# Autodesk Inventor assembly: ASY Disk Micro filter v2.0
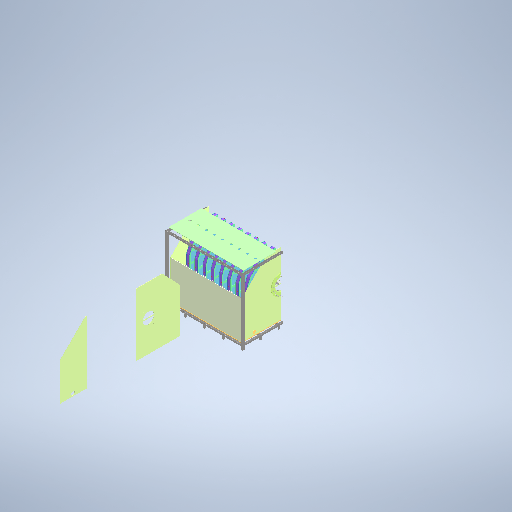
[picture p0: Inventor's stored thumbnail of the model, 512x512]
Saved by Autodesk Inventor 2025 (Build 290162010, 162A)
## iProperties
Created: 2023-08-31
Part Number: ASY Disk Micro filter v2.0
Document SubType Name: Assembly
Designer: admin
Stock Number: Дисковый_Фильтр
Author: admin
## Documents named in this file (29)
- C:\Users\pokla\Documents\Inventor\ДФО\ДМФ\DMF-Disk-Micro-Filter\ASY 000 ДМФ Disk Micro filter v2.0.iam
- C:\Users\pokla\Documents\Inventor\ДФО\ДМФ\DMF-Disk-Micro-Filter\Left wall v2.0.ipt
- C:\Users\pokla\Documents\Inventor\ДФО\ДМФ\DMF-Disk-Micro-Filter\Wall right v2.0.ipt
- C:\Users\pokla\Documents\Inventor\ДФО\ДМФ\DMF-Disk-Micro-Filter\DF1.03 Wall bottom v2.0.ipt
- C:\Users\pokla\Documents\Inventor\ДФО\ДМФ\DMF-Disk-Micro-Filter\DF1.04 Wall face v2.0.ipt
- C:\Users\pokla\Documents\Inventor\ДФО\ДМФ\DMF-Disk-Micro-Filter\ыASY xDF frame v2.0.iam
- C:\Users\pokla\Documents\Inventor\ДФО\ДМФ\DMF-Disk-Micro-Filter\ДМФ 021 кольцо прижимное нос v2.0.ipt
- C:\Users\pokla\Documents\Inventor\ДФО\ДМФ\DMF-Disk-Micro-Filter\ДМФ 000 размеры v2.0.ipt
- C:\Users\pokla\Documents\Inventor\ДФО\ДМФ\DMF-Disk-Micro-Filter\ASY ДМФ 030 кольцо со шпильками корма v2.0.iam
- C:\Users\pokla\Documents\Inventor\ДФО\ДМФ\DMF-Disk-Micro-Filter\ДМФ 032 крышка Нос v2.0.ipt
- C:\Users\pokla\Documents\Inventor\ДФО\ДМФ\DMF-Disk-Micro-Filter\ASY ДМФ 0100 Барабан v2.0.iam
- C:\Users\pokla\Documents\Inventor\ДФО\ДМФ\DMF-Disk-Micro-Filter\ДМФ 091 Постель НОС v2.0.ipt
- C:\Users\pokla\Documents\Inventor\ДФО\ДМФ\DMF-Disk-Micro-Filter\ASY ДМФ 040 кольцо под шпильки КОРМА v2.0.iam
- C:\Users\pokla\Documents\Inventor\ДФО\ДМФ\DMF-Disk-Micro-Filter\ДМФ 022 кольцо прижимное корма v2.0.ipt
- C:\Users\pokla\Documents\Inventor\ДФО\ДМФ\DMF-Disk-Micro-Filter\ДМФ 093 Постель КОРМА v2.0.ipt
- C:\Users\pokla\Documents\Inventor\ДФО\ДМФ\DMF-Disk-Micro-Filter\ДМФ 092 Коромысло КОРМА v2.0.ipt
- C:\Users\pokla\Documents\Inventor\ДФО\ДМФ\DMF-Disk-Micro-Filter\ДМФ 055 труба илоотвода v2.0.ipt
- C:\Users\pokla\Documents\Inventor\ДФО\ДМФ\DMF-Disk-Micro-Filter\ДМФ 033 держатель лотка v2.0.ipt
- C:\Users\pokla\Documents\Inventor\ДФО\ДМФ\DMF-Disk-Micro-Filter\ASY ДМФ лоток 050 илоотвод v2.0.iam
- C:\Users\pokla\Documents\Inventor\ДФО\ДМФ\DMF-Disk-Micro-Filter\ДМФ 092 Коромысло НОС v2.0.ipt
- C:\Users\pokla\Documents\Inventor\ДФО\ДМФ\DMF-Disk-Micro-Filter\ДМФ 011 Стенка Корма ЛЕВ v2.0.ipt
- C:\Users\pokla\Documents\Inventor\ДФО\ДМФ\DMF-Disk-Micro-Filter\ДМФ 012 Стенка Корма ПРАВ v2.0.ipt
- C:\Users\pokla\Documents\Inventor\ДФО\ДМФ\DMF-Disk-Micro-Filter\ДМФ 014 Стенка Нос ЛЕВ v2.0.ipt
- C:\Users\pokla\Documents\Inventor\ДФО\ДМФ\DMF-Disk-Micro-Filter\ДМФ 015 Стенка Нос ПРАВ v2.0.ipt
- C:\Users\pokla\Documents\Inventor\ДФО\ДМФ\DMF-Disk-Micro-Filter\ДМФ 066 Гребенка v2.0.ipt
- C:\Users\pokla\Documents\Inventor\ДФО\ДМФ\DMF-Disk-Micro-Filter\ДМФ 025 кольцо прижимное корма наружное v2.0.ipt
- C:\Users\pokla\Documents\Inventor\ДФО\ДМФ\DMF-Disk-Micro-Filter\ASY ДМФ 070 кольцо под шпильки КОРМА наружное v2.0.iam
- C:\Users\pokla\Documents\Inventor\ДФО\ДМФ\DMF-Disk-Micro-Filter\ДМФ 067 крышка v2.0.ipt
- C:\Users\pokla\Documents\Inventor\ДФО\ДМФ\DMF-Disk-Micro-Filter\ДМФ 081 труба форсунки v2.0.ipt
## Components (28 placed, 28 different names)
1. ДМФ 000 размеры v2.0.ipt:1
2. Left wall v2.0.ipt:1 — Flush:3, Flush:4, Mate:1, Flush:6, Flush:7, Flush:9, Mate:4, Flush:16, Rotational:12, Rigid:9, Rigid:12
3. Wall right v2.0.ipt:1 — Flush:3, Mate:2, Flush:8, Mate:22, Rigid:14, Flush:23, Flush:24
4. DF1.03 Wall bottom v2.0.ipt:1 — Mate:1, Mate:2, Flush:6, Flush:7, Flush:8, Mate:3, Flush:11, Mate:5, Mate:24
5. DF1.04 Wall face v2.0.ipt:1 — Flush:9, Mate:3, Mate:4, Flush:10, Angle:1
6. ыASY xDF frame v2.0.iam:1 [sub-assembly] — Flush:15, Flush:13, Flush:14, Mate:5
7. ДМФ 021 кольцо прижимное нос v2.0.ipt:1 — Rotational:12, Mate:13, Rotational:14
8. ASY ДМФ 030 кольцо со шпильками корма v2.0.iam:1 [sub-assembly] — Flush:16, Rigid:9
9. ДМФ 032 крышка Нос v2.0.ipt:1 — Mate:16, Rigid:8, Rigid:12
10. ASY ДМФ 0100 Барабан v2.0.iam:1 [sub-assembly] — Rotational:15
11. ДМФ 091 Постель НОС v2.0.ipt:1 — Flush:17, Rotational:14, Rigid:10, Rotational:15
12. ASY ДМФ 040 кольцо под шпильки КОРМА v2.0.iam:1 [sub-assembly] — Mate:14, Rigid:13
13. ДМФ 022 кольцо прижимное корма v2.0.ipt:1 — Flush:18, Rigid:11, Rigid:13
14. ДМФ 093 Постель КОРМА v2.0.ipt:1 — Mate:15, Rigid:3, Rigid:11
15. ДМФ 092 Коромысло КОРМА v2.0.ipt:1 — Rigid:3
16. ДМФ 055 труба илоотвода v2.0.ipt:1 — Rigid:8, Tangent:1
17. ДМФ 033 держатель лотка v2.0.ipt:1 — Mate:16, Mate:17, Tangent:1, Mate:23
18. ASY ДМФ лоток 050 илоотвод v2.0.iam:1 [sub-assembly] — Mate:22, Mate:23
19. ДМФ 092 Коромысло НОС v2.0.ipt:1 — Rigid:10
20. ДМФ 011 Стенка Корма ЛЕВ v2.0.ipt:1
21. ДМФ 012 Стенка Корма ПРАВ v2.0.ipt:1
22. ДМФ 014 Стенка Нос ЛЕВ v2.0.ipt:1
23. ДМФ 015 Стенка Нос ПРАВ v2.0.ipt:1
24. ДМФ 066 Гребенка v2.0.ipt:1 — Flush:22, Angle:1, Mate:24
25. ДМФ 025 кольцо прижимное корма наружное v2.0.ipt:1 — Rigid:14, Rigid:15
26. ASY ДМФ 070 кольцо под шпильки КОРМА наружное v2.0.iam:1 [sub-assembly] — Rigid:15
27. ДМФ 067 крышка v2.0.ipt:1 — Flush:23, Flush:24, Flush:25, Rotational:16
28. ДМФ 081 труба форсунки v2.0.ipt:1 — Flush:25, Rotational:16
## Relationships (48: Flush 19, Mate 14, WeldJoint 9, RevoluteJoint 4, Tangent 1, Angle 1)
- Flush:3: Left wall v2.0.ipt:1 ↔ Wall right v2.0.ipt:1
- Flush:4: Left wall v2.0.ipt:1
- Mate:1: Left wall v2.0.ipt:1 ↔ DF1.03 Wall bottom v2.0.ipt:1
- Mate:2: Wall right v2.0.ipt:1 ↔ DF1.03 Wall bottom v2.0.ipt:1
- Flush:6 (15 mm): Left wall v2.0.ipt:1 ↔ DF1.03 Wall bottom v2.0.ipt:1
- Flush:7 (25 mm): Left wall v2.0.ipt:1 ↔ DF1.03 Wall bottom v2.0.ipt:1
- Flush:8 (15 mm): Wall right v2.0.ipt:1 ↔ DF1.03 Wall bottom v2.0.ipt:1
- Flush:9: Left wall v2.0.ipt:1 ↔ DF1.04 Wall face v2.0.ipt:1
- Mate:3: DF1.03 Wall bottom v2.0.ipt:1 ↔ DF1.04 Wall face v2.0.ipt:1
- Mate:4: Left wall v2.0.ipt:1 ↔ DF1.04 Wall face v2.0.ipt:1
- Flush:10: DF1.04 Wall face v2.0.ipt:1
- Flush:11: DF1.03 Wall bottom v2.0.ipt:1
- [Flush]: ыASY xDF frame v2.0.iam:1
- Flush:15: ыASY xDF frame v2.0.iam:1
- Flush:13: ыASY xDF frame v2.0.iam:1
- Flush:14: ыASY xDF frame v2.0.iam:1
- Mate:5: DF1.03 Wall bottom v2.0.ipt:1 ↔ ыASY xDF frame v2.0.iam:1
- Flush:16: Left wall v2.0.ipt:1 ↔ ASY ДМФ 030 кольцо со шпильками корма v2.0.iam:1
- Rotational:12 [RevoluteJoint]: Left wall v2.0.ipt:1 ↔ ДМФ 021 кольцо прижимное нос v2.0.ipt:1
- Mate:13: ДМФ 021 кольцо прижимное нос v2.0.ipt:1
- Flush:17: ДМФ 091 Постель НОС v2.0.ipt:1
- Mate:14: ASY ДМФ 040 кольцо под шпильки КОРМА v2.0.iam:1
- Flush:18: ДМФ 022 кольцо прижимное корма v2.0.ipt:1
- Mate:15: ДМФ 093 Постель КОРМА v2.0.ipt:1
- Rigid:3 [WeldJoint]: ДМФ 093 Постель КОРМА v2.0.ipt:1 ↔ ДМФ 092 Коромысло КОРМА v2.0.ipt:1
- [Mate]: ASY ДМФ лоток 050 илоотвод v2.0.iam:1
- Mate:16: ДМФ 032 крышка Нос v2.0.ipt:1 ↔ ДМФ 033 держатель лотка v2.0.ipt:1
- Mate:17: ДМФ 033 держатель лотка v2.0.ipt:1
- Rigid:8 [WeldJoint]: ДМФ 032 крышка Нос v2.0.ipt:1 ↔ ДМФ 055 труба илоотвода v2.0.ipt:1
- Rigid:9 [WeldJoint]: Left wall v2.0.ipt:1 ↔ ASY ДМФ 030 кольцо со шпильками корма v2.0.iam:1
- Tangent:1: ДМФ 055 труба илоотвода v2.0.ipt:1 ↔ ДМФ 033 держатель лотка v2.0.ipt:1
- Mate:22: Wall right v2.0.ipt:1 ↔ ASY ДМФ лоток 050 илоотвод v2.0.iam:1
- Mate:23: ДМФ 033 держатель лотка v2.0.ipt:1 ↔ ASY ДМФ лоток 050 илоотвод v2.0.iam:1
- Rotational:14 [RevoluteJoint]: ДМФ 021 кольцо прижимное нос v2.0.ipt:1 ↔ ДМФ 091 Постель НОС v2.0.ipt:1
- Rigid:10 [WeldJoint]: ДМФ 091 Постель НОС v2.0.ipt:1 ↔ ДМФ 092 Коромысло НОС v2.0.ipt:1
- Rotational:15 [RevoluteJoint]: ASY ДМФ 0100 Барабан v2.0.iam:1 ↔ ДМФ 091 Постель НОС v2.0.ipt:1
- Rigid:11 [WeldJoint]: ДМФ 022 кольцо прижимное корма v2.0.ipt:1 ↔ ДМФ 093 Постель КОРМА v2.0.ipt:1
- Rigid:12 [WeldJoint]: Left wall v2.0.ipt:1 ↔ ДМФ 032 крышка Нос v2.0.ipt:1
- Flush:22: ДМФ 066 Гребенка v2.0.ipt:1
- Angle:1 (180 deg): DF1.04 Wall face v2.0.ipt:1 ↔ ДМФ 066 Гребенка v2.0.ipt:1
- Mate:24: DF1.03 Wall bottom v2.0.ipt:1 ↔ ДМФ 066 Гребенка v2.0.ipt:1
- Rigid:13 [WeldJoint]: ASY ДМФ 040 кольцо под шпильки КОРМА v2.0.iam:1 ↔ ДМФ 022 кольцо прижимное корма v2.0.ipt:1
- Rigid:14 [WeldJoint]: Wall right v2.0.ipt:1 ↔ ДМФ 025 кольцо прижимное корма наружное v2.0.ipt:1
- Rigid:15 [WeldJoint]: ДМФ 025 кольцо прижимное корма наружное v2.0.ipt:1 ↔ ASY ДМФ 070 кольцо под шпильки КОРМА наружное v2.0.iam:1
- Flush:23: Wall right v2.0.ipt:1 ↔ ДМФ 067 крышка v2.0.ipt:1
- Flush:24 (-50 mm): Wall right v2.0.ipt:1 ↔ ДМФ 067 крышка v2.0.ipt:1
- Flush:25: ДМФ 067 крышка v2.0.ipt:1 ↔ ДМФ 081 труба форсунки v2.0.ipt:1
- Rotational:16 [RevoluteJoint]: ДМФ 067 крышка v2.0.ipt:1 ↔ ДМФ 081 труба форсунки v2.0.ipt:1
